# Autodesk Inventor assembly: final_box_assembly
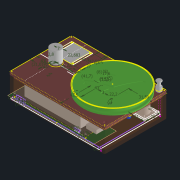
[picture p0: Inventor's stored thumbnail of the model, 180x180]
Saved by Autodesk Inventor 2021 (Build 250183000, 183)
## iProperties
Created: 2021-12-18
Part Number: final_box_assembly
Document SubType Name: Assembly
Designer: Juan M. Casillas
Author: Juan M. Casillas
## Documents named in this file (9)
- K:\3DPrinting\3DModels\3party\ElectricEel_rueca\medidor\v1\final_box_assembly.iam
- K:\3DPrinting\3DModels\3party\ElectricEel_rueca\medidor\battery_footprint.ipt
- K:\3DPrinting\3DModels\3party\ElectricEel_rueca\medidor\v1\assembly2.iam
- K:\3DPrinting\3DModels\3party\ElectricEel_rueca\medidor\encoder_footprint.ipt
- K:\3DPrinting\3DModels\3party\ElectricEel_rueca\medidor\buzzer_footprint.ipt
- K:\3DPrinting\3DModels\3party\ElectricEel_rueca\medidor\screen_footprint.ipt
- K:\3DPrinting\3DModels\3party\ElectricEel_rueca\medidor\nano_footprint.ipt
- K:\3DPrinting\3DModels\3party\ElectricEel_rueca\medidor\v1\box_final.ipt
- K:\3DPrinting\3DModels\3party\ElectricEel_rueca\medidor\v1\guia.ipt
## Components (8 placed, 8 different names)
1. battery_footprint:1 — Flush:1
2. assembly2:1 [sub-assembly]
3. encoder_footprint:1
4. buzzer_footprint:1
5. screen_footprint:1
6. nano_footprint:1
7. box_final:1
8. guia:1
## Relationships (1: Flush 1)
- Flush:1 (1 mm): battery_footprint:1
